# Autodesk Inventor assembly: PlanetaryGear
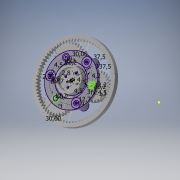
[picture p0: Inventor's stored thumbnail of the model, 180x180]
Saved by Autodesk Inventor 2018.3 (Build 223284000, 284)
## iProperties
Created: 2018-07-08
Part Number: PlanetaryGear
Material: Generisch
Document SubType Name: Assembly
Designer: JochenAlt
Author: JochenAlt
## Documents named in this file (8)
- D:\Projects\FlowerPot\CAD\PlanetaryGear\PlanetaryGear.iam
- D:\Projects\FlowerPot\CAD\PlanetaryGear\Konstruktions-Assistent\Stirnzahnrad21.ipt
- D:\Projects\FlowerPot\CAD\PlanetaryGear\Konstruktions-Assistent\Stirnzahnrad23.ipt
- D:\Projects\FlowerPot\CAD\PlanetaryGear\PlanetaryHolder.ipt
- D:\Projects\FlowerPot\CAD\PlanetaryGear\PlanetaryHolderTop.ipt
- D:\Projects\FlowerPot\CAD\Mounting Hub.ipt
- D:\Projects\FlowerPot\CAD\PlanetaryGear\PlanetaryHolderBottom.ipt
- D:\Projects\FlowerPot\CAD\PlanetaryGear\PlanetaryGearConstr\Konstruktions-Assistent\Stirnzahnrad12.ipt
## Components (9 placed, 6 different names)
1. Stirnzahnrad2:1 — Passend:11, Fluchtend:1
2. Stirnzahnrad2:2 — Passend:4, Passend:7, Fluchtend:1
3. Stirnzahnrad2:3 — Passend:3, Passend:8, Fluchtend:2
4. Stirnzahnrad2:4 — Passend:5, Passend:6
5. PlanetaryHolder:1
6. PlanetaryHolderTop:1 — Passend:1, Passend:2, Passend:3, Passend:4, Passend:5, Passend:6, Passend:7, Passend:8, Passend:10, Passend:11
7. Mounting Hub:1 — Passend:1, Passend:2, Passend:9
8. PlanetaryHolderBottom:1 — Passend:9, Passend:10, Passend:12
9. Stirnzahnrad1:1 — Passend:12, Fluchtend:2
## Relationships (14: Mate 12, Flush 2)
- Passend:1 [Mate]: PlanetaryHolderTop:1 ↔ Mounting Hub:1
- Passend:2 [Mate]: PlanetaryHolderTop:1 ↔ Mounting Hub:1
- Passend:3 [Mate]: Stirnzahnrad2:3 ↔ PlanetaryHolderTop:1
- Passend:4 [Mate]: Stirnzahnrad2:2 ↔ PlanetaryHolderTop:1
- Passend:5 [Mate]: Stirnzahnrad2:4 ↔ PlanetaryHolderTop:1
- Passend:6 [Mate] (4 mm): Stirnzahnrad2:4 ↔ PlanetaryHolderTop:1
- Passend:7 [Mate] (4 mm): Stirnzahnrad2:2 ↔ PlanetaryHolderTop:1
- Passend:8 [Mate] (4 mm): Stirnzahnrad2:3 ↔ PlanetaryHolderTop:1
- Passend:9 [Mate]: Mounting Hub:1 ↔ PlanetaryHolderBottom:1
- Passend:10 [Mate]: PlanetaryHolderTop:1 ↔ PlanetaryHolderBottom:1
- Passend:11 [Mate]: Stirnzahnrad2:1 ↔ PlanetaryHolderTop:1
- Fluchtend:1 [Flush]: Stirnzahnrad2:1 ↔ Stirnzahnrad2:2
- Passend:12 [Mate]: PlanetaryHolderBottom:1 ↔ Stirnzahnrad1:1
- Fluchtend:2 [Flush]: Stirnzahnrad2:3 ↔ Stirnzahnrad1:1
